# Autodesk Inventor assembly: manipulator
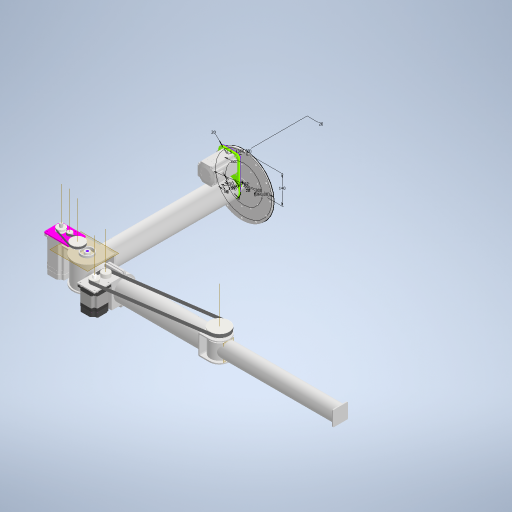
[picture p0: Inventor's stored thumbnail of the model, 512x512]
Saved by Autodesk Inventor 2023 (Build 270158000, 158)
## iProperties
Created: 2023-03-28
Part Number: manipulator
Document SubType Name: Assembly
Designer: krzys
Author: krzys
## Documents named in this file (17)
- C:\Users\krzys\Documents\GitHub\Manipulator-Inventor\Manipulator.iam
- C:\Users\krzys\Documents\GitHub\Manipulator-Inventor\podstawa.ipt
- C:\Users\krzys\Documents\GitHub\Manipulator-Inventor\manipulator\Design Accelerator\Łożysko1.iam
- C:\Users\krzys\Documents\GitHub\Manipulator-Inventor\tuleja_dystansowa.ipt
- C:\Users\krzys\Documents\GitHub\Manipulator-Inventor\podstwa_obrotowa.ipt
- C:\Users\krzys\Documents\GitHub\Manipulator-Inventor\CS-M23480_3D.ipt
- C:\Users\krzys\Documents\GitHub\Manipulator-Inventor\czlon 1 i 2.iam
- C:\Users\krzys\Documents\GitHub\Manipulator-Inventor\Manipulator\Design Accelerator\Łożysko6.iam
- C:\Users\krzys\Documents\GitHub\Manipulator-Inventor\Wał2.ipt
- C:\Users\krzys\Documents\GitHub\Manipulator-Inventor\Manipulator\Design Accelerator\Przekładnie walcowe1.iam
- C:\Users\krzys\Documents\GitHub\Manipulator-Inventor\czlon 3.ipt
- C:\Users\krzys\Documents\GitHub\Manipulator-Inventor\mocowanie silnika.ipt
- C:\Users\krzys\Documents\GitHub\Manipulator-Inventor\silniki\CS-M23485B_3D.ipt
- C:\Users\krzys\Documents\GitHub\Manipulator-Inventor\Manipulator\Design Accelerator\Przekładnie pasowe synchroniczne1.iam
- C:\Users\krzys\Documents\GitHub\Manipulator-Inventor\silniki\mocowanie_silnika_członu_3.ipt
- C:\Users\krzys\Documents\GitHub\Manipulator-Inventor\silniki\CS-M23445WP_3D.iam
- C:\Users\krzys\Documents\GitHub\Manipulator-Inventor\Manipulator\Design Accelerator\Przekładnie pasowe synchroniczne2.iam
## Components (17 placed, 14 different names)
1. podstawa:1
2. Łożysko:1 [sub-assembly]
3. Łożysko:2 [sub-assembly]
4. tuleja_dystansowa:1
5. podstwa_obrotowa:1 — Zestawiające:2, Zestawiające:3
6. CS-M23480_3D:1 — Zestawiające:2
7. czlon 1 i 2:1 [sub-assembly] — Zestawiające:3, Wstawiające:1, Zestawiające:6, Wstawiające:2, Równoległe:4, Równoległe:5, Wstawiające:4
8. Łożysko:3 [sub-assembly] — Wstawiające:1, Zestawiające:4, Równoległe:1, Kątowe:1
9. Wał:1 — Zestawiające:4, Równoległe:1, Kątowe:1, Zestawiające:5, Równoległe:2, Równoległe:3
10. Przekładnie walcowe:1 [sub-assembly] — Zestawiające:5, Równoległe:2, Zestawiające:6, Równoległe:3
11. czlon 3:1 — Wstawiające:2
12. mocowanie silnika:1 — Równoległe:4, Równoległe:5, Wstawiające:3
13. CS-M23485B_3D:1 — Wstawiające:3
14. Przekładnie pasowe synchroniczne:1 [sub-assembly]
15. mocowanie_silnika_członu_3:1 — Wstawiające:4, Wstawiające:5
16. CS-M23445WP_3D:1 [sub-assembly] — Wstawiające:5
17. Przekładnie pasowe synchroniczne:2 [sub-assembly]
## Relationships (16: Mate 5, Insert 5, Flush 5, Angle 1)
- Zestawiające:2 [Mate]: podstwa_obrotowa:1 ↔ CS-M23480_3D:1
- Zestawiające:3 [Mate]: podstwa_obrotowa:1 ↔ czlon 1 i 2:1
- Wstawiające:1 [Insert]: czlon 1 i 2:1 ↔ Łożysko:3
- Zestawiające:4 [Mate]: Łożysko:3 ↔ Wał:1
- Równoległe:1 [Flush] (-15 mm): Łożysko:3 ↔ Wał:1
- Kątowe:1 [Angle] (0 deg): Łożysko:3 ↔ Wał:1
- Zestawiające:5 [Mate]: Wał:1 ↔ Przekładnie walcowe:1
- Równoległe:2 [Flush]: Wał:1 ↔ Przekładnie walcowe:1
- Zestawiające:6 [Mate]: czlon 1 i 2:1 ↔ Przekładnie walcowe:1
- Równoległe:3 [Flush]: Wał:1 ↔ Przekładnie walcowe:1
- Wstawiające:2 [Insert] (13.5 mm): czlon 1 i 2:1 ↔ czlon 3:1
- Równoległe:4 [Flush]: czlon 1 i 2:1 ↔ mocowanie silnika:1
- Równoległe:5 [Flush]: czlon 1 i 2:1 ↔ mocowanie silnika:1
- Wstawiające:3 [Insert]: mocowanie silnika:1 ↔ CS-M23485B_3D:1
- Wstawiające:4 [Insert] (-500 mm): czlon 1 i 2:1 ↔ mocowanie_silnika_członu_3:1
- Wstawiające:5 [Insert]: mocowanie_silnika_członu_3:1 ↔ CS-M23445WP_3D:1
